# Autodesk Inventor assembly: controler
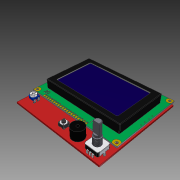
[picture p0: Inventor's stored thumbnail of the model, 180x180]
Saved by Autodesk Inventor 2014 (Build 180170000, 170)
## iProperties
Created: 2014-03-22
Part Number: controler
Document SubType Name: Assembly
Designer: buben
Author: buben
## Documents named in this file (8)
- C:\Users\buben\Documents\GitHub\bacon\inventor files\utils\ramps_smart_controller\controler.iam
- C:\Users\buben\Documents\GitHub\bacon\inventor files\3rd party components\128x64_matrix_lcd\Imported Components\RG12864A-BIY-V\RG12864A-BIY-V.ipt
- C:\Users\buben\Documents\GitHub\bacon\inventor files\utils\ramps_smart_controller\motherboard_pcb.ipt
- C:\Users\buben\Documents\GitHub\bacon\inventor files\3rd party components\rotary_encoder\12mm Incremental Encoder - BOURNS PEC11S.iam
- C:\Users\buben\Documents\GitHub\bacon\inventor files\utils\ramps_smart_controller\piezo_buzzer.ipt
- C:\Users\buben\Documents\GitHub\bacon\inventor files\3rd party components\tactileswitch-short\Imported Components\tactileswitch-short\tactileswitch-short.ipt
- C:\Users\buben\Documents\GitHub\bacon\inventor files\3rd party components\potentiometer\Imported Components\Pot - RES_VAR1\Pot - RES_VAR1.ipt
- C:\Users\buben\Documents\GitHub\bacon\inventor files\3rd party components\sd_card\Imported Components\SD\SD.ipt
## Components (7 placed, 7 different names)
1. RG12864A-BIY-V:1 — Mate:1, Flush:1, Flush:2
2. motherboard_pcb:1 — Mate:1, Flush:1, Flush:2, Mate:2, Mate:3, Mate:4, Mate:5, Flush:3, Flush:4, Mate:6, Mate:7, Angle:1, Mate:8, Mate:9, Angle:2, Flush:5, Flush:6, Mate:10, Mate:14, Flush:7, Flush:8
3. 12mm Incremental Encoder - BOURNS PEC11S:1 [sub-assembly] — Mate:2, Mate:6, Mate:7, Angle:1, Mate:13
4. piezo_buzzer:1 — Mate:3, Mate:8, Mate:12, Mate:13
5. tactileswitch-short:1 — Mate:4, Mate:9, Angle:2, Mate:12
6. Pot - RES_VAR1:1 — Mate:5, Flush:3, Flush:4
7. SD:1 — Mate:14, Flush:7, Flush:8
## Relationships (23: Mate 13, Flush 8, Angle 2)
- Mate:1 (2.8 mm): RG12864A-BIY-V:1 ↔ motherboard_pcb:1
- Flush:1: RG12864A-BIY-V:1 ↔ motherboard_pcb:1
- Flush:2: RG12864A-BIY-V:1 ↔ motherboard_pcb:1
- Mate:2 (2 mm): motherboard_pcb:1 ↔ 12mm Incremental Encoder - BOURNS PEC11S:1
- Mate:3: motherboard_pcb:1 ↔ piezo_buzzer:1
- Mate:4: motherboard_pcb:1 ↔ tactileswitch-short:1
- Mate:5: motherboard_pcb:1 ↔ Pot - RES_VAR1:1
- Flush:3 (-8 mm): motherboard_pcb:1 ↔ Pot - RES_VAR1:1
- Flush:4 (5.5 mm): motherboard_pcb:1 ↔ Pot - RES_VAR1:1
- Mate:6 (-10 mm): motherboard_pcb:1 ↔ 12mm Incremental Encoder - BOURNS PEC11S:1
- Mate:7 (-8.5 mm): motherboard_pcb:1 ↔ 12mm Incremental Encoder - BOURNS PEC11S:1
- Angle:1 (0 deg): motherboard_pcb:1 ↔ 12mm Incremental Encoder - BOURNS PEC11S:1
- Mate:8 (-8.5 mm): motherboard_pcb:1 ↔ piezo_buzzer:1
- Mate:9 (-8.5 mm): motherboard_pcb:1 ↔ tactileswitch-short:1
- Angle:2 (0 deg): motherboard_pcb:1 ↔ tactileswitch-short:1
- Flush:5: motherboard_pcb:1
- Flush:6: motherboard_pcb:1
- Mate:10: motherboard_pcb:1
- Mate:12 (15.175 mm): piezo_buzzer:1 ↔ tactileswitch-short:1
- Mate:13 (18.75 mm): 12mm Incremental Encoder - BOURNS PEC11S:1 ↔ piezo_buzzer:1
- Mate:14 (0.5 mm): motherboard_pcb:1 ↔ SD:1
- Flush:7 (23.5 mm): motherboard_pcb:1 ↔ SD:1
- Flush:8 (-10.5 mm): motherboard_pcb:1 ↔ SD:1
